# Autodesk Inventor assembly: kayboard
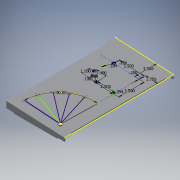
[picture p0: Inventor's stored thumbnail of the model, 180x180]
Saved by Autodesk Inventor 2016 SP2 (Build 200236200, 236)
## iProperties
Created: 2017-09-03
Part Number: kayboard
Document SubType Name: Assembly
Designer: Kartikye
Author: Kartikye
## Documents named in this file (4)
- D:\Documents\cs294\keyboard\kayboard.iam
- D:\Documents\cs294\keyboard\main board.ipt
- D:\Documents\cs294\keyboard\swiweller.ipt
- D:\Documents\cs294\keyboard\side board.ipt
## Components (4 placed, 3 different names)
1. swiweller:1 — Insert:1
2. main board:1 — Insert:1, Mate:1, Flush:1, Mate:2, Mate:3, Flush:2, Mate:4
3. side board:1 — Mate:1, Flush:1, Mate:2
4. side board:2 — Mate:3, Flush:2, Mate:4
## Relationships (7: Mate 4, Flush 2, Insert 1)
- Insert:1: swiweller:1 ↔ main board:1
- Mate:1: main board:1 ↔ side board:1
- Flush:1: main board:1 ↔ side board:1
- Mate:2: main board:1 ↔ side board:1
- Mate:3: main board:1 ↔ side board:2
- Flush:2: main board:1 ↔ side board:2
- Mate:4: main board:1 ↔ side board:2
